# Autodesk Inventor assembly: Core
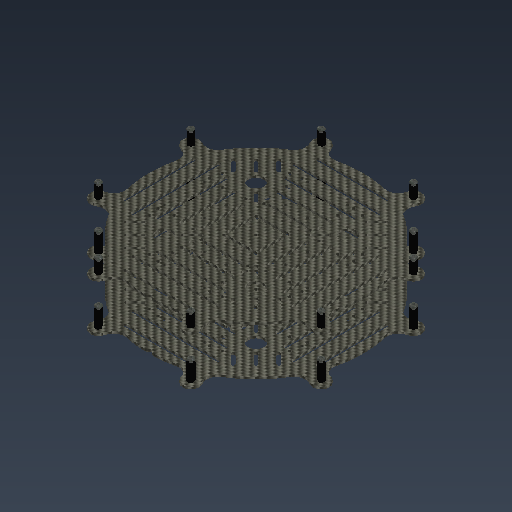
[picture p0: Inventor's stored thumbnail of the model, 512x512]
Saved by Autodesk Inventor 2024.1 (Build 281209000, 209)
## iProperties
Created: 2023-12-05
Part Number: Core
Document SubType Name: Assembly
Designer: dzw04
Mass: 217.944 g
Surface Area: 1420.64 cm^2
Volume: 117.544 cm^3
Density: 1.85414 g/cm^3
Author: dzw04
## Documents named in this file (6)
- C:\Users\dzw04\Saxion\Mechatronica Lectoraat LMECH LED - Database ARG\Component_Database\SARAX\01. CAD\01. 3D_Drawing\02. Sub_Assemblies\Core\Core.iam
- C:\Users\dzw04\Saxion\Mechatronica Lectoraat LMECH LED - Database ARG\Component_Database\SARAX\01. CAD\01. 3D_Drawing\02. Sub_Assemblies\Core\01. Parts\Body_Center_Plate.ipt
- C:\Users\dzw04\Saxion\Mechatronica Lectoraat LMECH LED - Database ARG\Component_Database\SARAX\01. CAD\01. 3D_Drawing\01. Parts\Standoff_M3_10mm.ipt
- C:\Users\dzw04\Saxion\Mechatronica Lectoraat LMECH LED - Database ARG\Component_Database\SARAX\01. CAD\01. 3D_Drawing\01. Parts\en-US\ISO 7380-1\ISO 7380-1 - M3 x 6.ipt
- C:\Users\dzw04\Saxion\Mechatronica Lectoraat LMECH LED - Database ARG\Component_Database\SARAX\01. CAD\01. 3D_Drawing\01. Parts\Standoff_M3_15mm.ipt
- C:\Users\dzw04\Saxion\Mechatronica Lectoraat LMECH LED - Database ARG\Component_Database\SARAX\01. CAD\01. 3D_Drawing\Parameters.xlsx
## Components (50 placed, 4 different names)
1. Body_Center_Plate:1 — Mate:1, Mate:2, Mate:3, Mate:8, Mate:9
2. Body_Center_Plate:2 — Mate:1, Mate:2, Mate:3, Mate:4, Mate:5
3. Standoff_M3_10mm:1 — Mate:4, Mate:5, Mate:6, Mate:7, Mate:12, Mate:13
4. ISO 7380-1 M3 x 6:1 — Mate:12, Mate:13
5. ISO 7380-1 M3 x 6:2 — Mate:6, Mate:7
6. Standoff_M3_10mm:2
7. ISO 7380-1 M3 x 6:3
8. ISO 7380-1 M3 x 6:4
9. Standoff_M3_10mm:3
10. ISO 7380-1 M3 x 6:5
11. ISO 7380-1 M3 x 6:6
12. Standoff_M3_10mm:4
13. ISO 7380-1 M3 x 6:7
14. ISO 7380-1 M3 x 6:8
15. Standoff_M3_10mm:5
16. ISO 7380-1 M3 x 6:9
17. ISO 7380-1 M3 x 6:10
18. Standoff_M3_10mm:6
19. ISO 7380-1 M3 x 6:11
20. ISO 7380-1 M3 x 6:12
21. Standoff_M3_10mm:7
22. ISO 7380-1 M3 x 6:13
23. ISO 7380-1 M3 x 6:14
24. Standoff_M3_10mm:8
25. ISO 7380-1 M3 x 6:15
26. ISO 7380-1 M3 x 6:16
27. Standoff_M3_15mm:1 — Mate:8, Mate:9, Mate:10, Mate:11, Mate:14, Mate:15
28. ISO 7380-1 M3 x 6:17 — Mate:14, Mate:15
29. ISO 7380-1 M3 x 6:18 — Mate:10, Mate:11
30. Standoff_M3_15mm:2
31. ISO 7380-1 M3 x 6:19
32. ISO 7380-1 M3 x 6:20
33. Standoff_M3_15mm:3
34. ISO 7380-1 M3 x 6:21
35. ISO 7380-1 M3 x 6:22
36. Standoff_M3_15mm:4
37. ISO 7380-1 M3 x 6:23
38. ISO 7380-1 M3 x 6:24
39. Standoff_M3_15mm:5
40. ISO 7380-1 M3 x 6:25
41. ISO 7380-1 M3 x 6:26
42. Standoff_M3_15mm:6
43. ISO 7380-1 M3 x 6:27
44. ISO 7380-1 M3 x 6:28
45. Standoff_M3_15mm:7
46. ISO 7380-1 M3 x 6:29
47. ISO 7380-1 M3 x 6:30
48. Standoff_M3_15mm:8
49. ISO 7380-1 M3 x 6:31
50. ISO 7380-1 M3 x 6:32
## Component patterns: (8 elements, first: Standoff_M3_10mm:1 + ISO 7380-1 M3 x 6:1 + ISO 7380-1 M3 x 6:2), (8 elements, first: Standoff_M3_15mm:1 + ISO 7380-1 M3 x 6:17 + ISO 7380-1 M3 x 6:18)
## Relationships (15: Mate 15)
- Mate:1 (42 mm): Body_Center_Plate:1 ↔ Body_Center_Plate:2
- Mate:2: Body_Center_Plate:1 ↔ Body_Center_Plate:2
- Mate:3: Body_Center_Plate:1 ↔ Body_Center_Plate:2
- Mate:4: Body_Center_Plate:2 ↔ Standoff_M3_10mm:1
- Mate:5: Body_Center_Plate:2 ↔ Standoff_M3_10mm:1
- Mate:6 (2 mm): Standoff_M3_10mm:1 ↔ ISO 7380-1 M3 x 6:2
- Mate:7: Standoff_M3_10mm:1 ↔ ISO 7380-1 M3 x 6:2
- Mate:8: Body_Center_Plate:1 ↔ Standoff_M3_15mm:1
- Mate:9: Body_Center_Plate:1 ↔ Standoff_M3_15mm:1
- Mate:10 (2 mm): Standoff_M3_15mm:1 ↔ ISO 7380-1 M3 x 6:18
- Mate:11: Standoff_M3_15mm:1 ↔ ISO 7380-1 M3 x 6:18
- Mate:12 (2 mm): Standoff_M3_10mm:1 ↔ ISO 7380-1 M3 x 6:1
- Mate:13: Standoff_M3_10mm:1 ↔ ISO 7380-1 M3 x 6:1
- Mate:14 (2 mm): Standoff_M3_15mm:1 ↔ ISO 7380-1 M3 x 6:17
- Mate:15: Standoff_M3_15mm:1 ↔ ISO 7380-1 M3 x 6:17
## Named parameters: NumberOfArms = 4, RotorToRotor = 900 mm, MountToMotorCenter = 0 mm, ArmPosition = 5 deg, LoadpipeLength = 450 mm, LandingGearHeight = 400 mm, NumberOfBatterys = 2, BatteryLength = 200 mm, BatteryWidth = 62 mm, BatteryHeight = 76 mm, ThicknessBodyOuterPlate = 2 mm, ThicknessBodyCenterPlate = 2 mm, ThicknessLegLoadpipePlate = 2 mm, ThicknessBatteryTray = 2 mm, ThicknessBatteryTopTray = 1 mm, LandingGearRod = 390 mm, LandingGearStabilityBar = 525 mm, StartAngleArm = 45 deg, MotorMountCenter = 71.5 mm
